# Autodesk Inventor assembly: TankFlipper
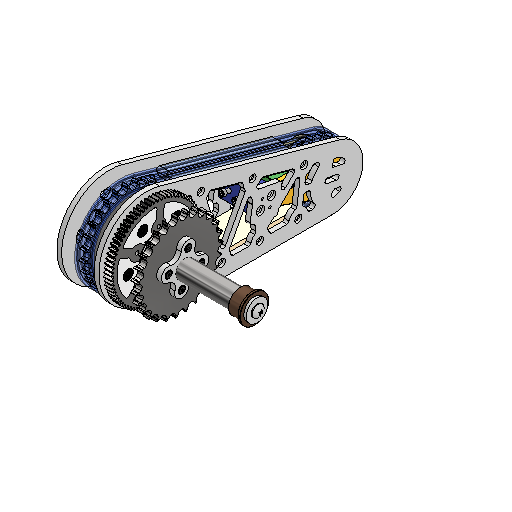
[picture p0: Inventor's stored thumbnail of the model, 512x512]
Saved by Autodesk Inventor 2025 (Build 290162000, 162)
## iProperties
Created: 2024-02-14
Part Number: TankFlipper
Document SubType Name: Assembly
Designer: seene
Author: seene
## Documents named in this file (9)
- C:\Users\seene\Desktop\Stony Brook\SBRT\RCR_Dexter\Drive\v1\TankFlipper Flipped.iam
- C:\Users\seene\Desktop\Stony Brook\SBRT\RCR_Dexter\Drive\v1\TANK flipper\panel_outside.ipt
- C:\Users\seene\Desktop\Stony Brook\SBRT\RCR_Dexter\Drive\v1\TANK flipper\panel_inside.ipt
- C:\Users\seene\Desktop\Stony Brook\SBRT\RCR_Dexter\Drive\v1\TANK flipper\flat chain guide.ipt
- C:\Users\seene\Desktop\Stony Brook\SBRT\RCR_Dexter\Drive\v1\TANK flipper\chain guide.ipt
- C:\Users\seene\Desktop\Stony Brook\SBRT\RCR_Dexter\Drive\v1\TANK flipper\TankFlipperAssembledDriveShaft.iam
- C:\Users\seene\Desktop\Stony Brook\SBRT\RCR_Dexter\Drive\v1\TANK flipper\flipper_tensioner _belt.iam
- C:\Users\seene\Desktop\Stony Brook\SBRT\RCR_Dexter\Drive\v1\TANK flipper\.25-20_FHCS_91263A553.ipt
- C:\Users\seene\Desktop\Stony Brook\SBRT\RCR_Dexter\Drive\v1\TankFlipper Flipped\Design Accelerator\Chain Drive1.iam
## Components (8 placed, 8 different names)
1. panel_outside:1 — Mate:1, Mate:2, Mate:3
2. panel_inside:1 — Mate:4, Mate:5, Mate:6, Mate:9, Mate:10, Rigid:1, Mate:11, Mate:12, Mate:13
3. flat chain guide:1 — Mate:1, Mate:2, Mate:3, Mate:4, Mate:5, Mate:10
4. chain guide:1 — Mate:6, Mate:9
5. TankFlipperAssembledDriveShaft:1 [sub-assembly] — Rigid:1
6. flipper_tensioner _belt:1 [sub-assembly] — Mate:11, Mate:12, Mate:13
7. .25-20_FHCS_91263A553:1
8. Chain Drive:1 [sub-assembly]
## Relationships (12: Mate 11, WeldJoint 1)
- Mate:1: panel_outside:1 ↔ flat chain guide:1
- Mate:2: panel_outside:1 ↔ flat chain guide:1
- Mate:3: panel_outside:1 ↔ flat chain guide:1
- Mate:4: panel_inside:1 ↔ flat chain guide:1
- Mate:5: panel_inside:1 ↔ flat chain guide:1
- Mate:6: panel_inside:1 ↔ chain guide:1
- Mate:9: panel_inside:1 ↔ chain guide:1
- Mate:10: panel_inside:1 ↔ flat chain guide:1
- Rigid:1 [WeldJoint]: panel_inside:1 ↔ TankFlipperAssembledDriveShaft:1
- Mate:11: panel_inside:1 ↔ flipper_tensioner _belt:1
- Mate:12: panel_inside:1 ↔ flipper_tensioner _belt:1
- Mate:13: panel_inside:1 ↔ flipper_tensioner _belt:1
